# Autodesk Inventor assembly: AXI 2204 Multicopter
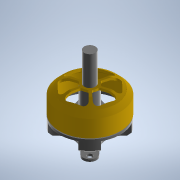
[picture p0: Inventor's stored thumbnail of the model, 180x180]
Saved by Autodesk Inventor 2021 (Build 250183000, 183)
## iProperties
Created: 2018-12-11
Part Number: AXI 2204 Multicopter
Document SubType Name: Assembly
Designer: Kanenas
Mass: 24 g
Surface Area: 50.333 cm^2
Volume: 2.84875 cm^3
Author: Kanenas
## Documents named in this file (3)
- E:\EPFL_MASTER\Sem proj\IISRD_CAD_V_v2\IISRD_V_v1\Motor_AXI_220454_GOLD_LINE_V2\AXI 2204 Multicopter.iam
- E:\EPFL_MASTER\Sem proj\IISRD_CAD_V_v2\IISRD_V_v1\Motor_AXI_220454_GOLD_LINE_V2\Motor Bot.ipt
- E:\EPFL_MASTER\Sem proj\IISRD_CAD_V_v2\IISRD_V_v1\Motor_AXI_220454_GOLD_LINE_V2\Motor Top.ipt
## Components (2 placed, 2 different names)
1. Motor Bot:1 — Mate:1, Mate:2
2. Motor Top:1 — Mate:1, Mate:2
## Relationships (2: Mate 2)
- Mate:1: Motor Bot:1 ↔ Motor Top:1
- Mate:2 (-17.97 mm): Motor Bot:1 ↔ Motor Top:1
